# Autodesk Inventor assembly: 3DrumWChain
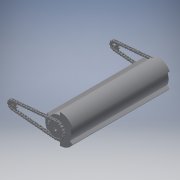
[picture p0: Inventor's stored thumbnail of the model, 180x180]
Saved by Autodesk Inventor 2016 (Build 200138000, 138)
## iProperties
Created: 2016-10-21
Part Number: 3DrumWChain
Document SubType Name: Assembly
Designer: Kevin
Author: Kevin
## Documents named in this file (5)
- C:\Users\Kevin\Documents\College\Senior Design\Drum spinner\3DrumWChain.iam
- C:\Users\Kevin\Documents\College\Senior Design\Drum spinner\Three_edge_drum.ipt
- C:\Users\Kevin\Downloads\sprocket19teeth.ipt
- C:\Users\Kevin\Downloads\sprocket9teeth.ipt
- C:\Users\Kevin\Documents\College\Senior Design\Chains\492RollerChain.iam
## Components (7 placed, 4 different names)
1. Three_edge_drum:1 — Mate:1
2. sprocket19teeth:1 — Mate:1
3. sprocket19teeth:2
4. sprocket9teeth:1
5. sprocket9teeth:2
6. 492RollerChain:1 [sub-assembly]
7. 492RollerChain:2 [sub-assembly]
## Relationships (1: Mate 1)
- Mate:1: Three_edge_drum:1 ↔ sprocket19teeth:1
